# Autodesk Inventor assembly: Estrutura ax
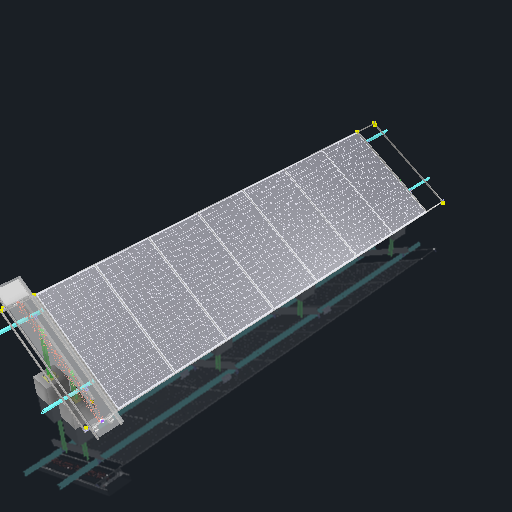
[picture p0: Inventor's stored thumbnail of the model, 512x512]
Saved by Autodesk Inventor 2025.3 (Build 293356030, 356C)
## iProperties
Created: 2019-12-15
Part Number: Estrutura ax
Document SubType Name: Assembly
Designer: Rubens
Sending System: SolidWorks 2021
Last Author: Mohsen
Last Saved: 2022-08-25
Author: Rubens
## Documents named in this file (17)
- C:\Users\Rubens\Downloads\Estrutura Placa - REV00\Solar Mounting Structure\Main_Solar_Structure\Main_Solar_Structure\Estrutura ax.iam
- C:\Users\Rubens\Downloads\Estrutura Placa - REV00\Solar Mounting Structure\Main_Solar_Structure\Main_Solar_Structure\Small_Column.ipt
- C:\Users\Rubens\Downloads\Estrutura Placa - REV00\Solar Mounting Structure\Main_Solar_Structure\Main_Solar_Structure\Large_Column.ipt
- C:\Users\Rubens\Downloads\Estrutura Placa - REV00\Solar Mounting Structure\Main_Solar_Structure\Main_Solar_Structure\Bottom_Beam.ipt
- C:\Users\Rubens\Downloads\Estrutura Placa - REV00\Solar Mounting Structure\Main_Solar_Structure\Main_Solar_Structure\Top_Beam.iam
- C:\Users\Rubens\Downloads\Estrutura Placa - REV00\Solar Mounting Structure\Main_Solar_Structure\Main_Solar_Structure\Base_Plate.ipt
- C:\Users\Rubens\Downloads\Estrutura Placa - REV00\Solar Mounting Structure\Main_Solar_Structure\Main_Solar_Structure\Base_Support.ipt
- C:\Users\Rubens\Downloads\Estrutura Placa - REV00\Solar Mounting Structure\Main_Solar_Structure\Main_Solar_Structure\Beam_Support.ipt
- C:\Users\Rubens\Downloads\Estrutura Placa - REV00\Solar Mounting Structure\Main_Solar_Structure\Main_Solar_Structure\M10_Screw&Nut.iam
- C:\Users\Rubens\Downloads\Estrutura Placa - REV00\Solar Mounting Structure\Main_Solar_Structure\Main_Solar_Structure\Beam_Connector_Assembly.iam
- C:\Users\Rubens\Downloads\Estrutura Placa - REV00\Solar Mounting Structure\Main_Solar_Structure\Main_Solar_Structure\Base.ipt
- C:\Users\Rubens\Downloads\Estrutura Placa - REV00\Solar Mounting Structure\Main_Solar_Structure\Main_Solar_Structure\ISO - 4034 - M16 - S_.ipt
- C:\Users\Rubens\Downloads\Limpador\MontagemREV0.iam
- C:\Users\Rubens\Downloads\Estrutura Placa - REV00\Solar Mounting Structure\Main_Solar_Structure\Main_Solar_Structure\SolarPV.ipt
- C:\Users\Rubens\Downloads\Estrutura Placa - REV00\Solar Mounting Structure\Main_Solar_Structure\Main_Solar_Structure\Perfil tubo - 30x30x3.ipt
- C:\Users\Rubens\Downloads\Estrutura Placa - REV00\Solar Mounting Structure\Main_Solar_Structure\Main_Solar_Structure\tubo 30 x 30 x 3  - 500.ipt
- C:\Users\Rubens\Downloads\Estrutura Placa - REV00\Solar Mounting Structure\Main_Solar_Structure\Main_Solar_Structure\Limitador.ipt
## Components (127 placed, 16 different names)
1. Small_Column:1 — Coincidente:18
2. Large_Column:1 — Coincidente:18
3. Bottom_Beam:1 — Coincidente:31, Coincidente:32, Coincidente:34
4. Bottom_Beam:2
5. Small_Column:2
6. Bottom_Beam:3
7. Small_Column:3
8. Bottom_Beam:4 — Coincidente:44, Coincidente:59
9. Small_Column:4
10. Top_Beam:3 [sub-assembly] — Coincidente:1, Coincidente:2, Coincidente:3, Coincidente:4, Coincidente:33, Alinhado:6, Coincidente:45
11. Top_Beam:4 [sub-assembly] — Coincidente:5, Coincidente:31, Coincidente:35, Alinhado:6, Coincidente:58
12. Base_Plate:1 — Coincidente:15
13. Base_Plate:2 — Coincidente:15, Coincidente:16, Coincidente:17
14. Base_Plate:4
15. Base_Plate:6
16. Base_Plate:8
17. Base_Support:1
18. Base_Support:2
19. Base_Support:3
20. Base_Support:7
21. Base_Support:8
22. Base_Support:9
23. Base_Support:13
24. Base_Support:14
25. Base_Support:15
26. Base_Support:19
27. Base_Support:20
28. Base_Support:21
29. Beam_Support:3 — Coincidente:32, Coincidente:33
30. Beam_Support:4 — Coincidente:34, Coincidente:35
31. Beam_Support:5
32. Beam_Support:6
33. Beam_Support:9
34. Beam_Support:10
35. M10_Screw&Nut:2 [sub-assembly]
36. M10_Screw&Nut:7 [sub-assembly]
37. M10_Screw&Nut:8 [sub-assembly]
38. M10_Screw&Nut:9 [sub-assembly]
39. M10_Screw&Nut:10 [sub-assembly]
40. M10_Screw&Nut:11 [sub-assembly]
41. M10_Screw&Nut:12 [sub-assembly]
42. M10_Screw&Nut:17 [sub-assembly]
43. M10_Screw&Nut:18 [sub-assembly]
44. M10_Screw&Nut:19 [sub-assembly]
45. M10_Screw&Nut:20 [sub-assembly]
46. M10_Screw&Nut:25 [sub-assembly]
47. M10_Screw&Nut:26 [sub-assembly]
48. M10_Screw&Nut:27 [sub-assembly]
49. M10_Screw&Nut:28 [sub-assembly]
50. M10_Screw&Nut:33 [sub-assembly]
51. M10_Screw&Nut:58 [sub-assembly] — Coincidente:62
52. M10_Screw&Nut:59 [sub-assembly] — Coincidente:63
53. M10_Screw&Nut:60 [sub-assembly]
54. M10_Screw&Nut:61 [sub-assembly]
55. M10_Screw&Nut:62 [sub-assembly]
56. M10_Screw&Nut:63 [sub-assembly]
57. M10_Screw&Nut:64 [sub-assembly]
58. M10_Screw&Nut:65 [sub-assembly]
59. M10_Screw&Nut:66 [sub-assembly]
60. M10_Screw&Nut:67 [sub-assembly]
61. M10_Screw&Nut:68 [sub-assembly]
62. M10_Screw&Nut:69 [sub-assembly]
63. M10_Screw&Nut:71 [sub-assembly] — Coincidente:60
64. M10_Screw&Nut:72 [sub-assembly] — Coincidente:61
65. M10_Screw&Nut:73 [sub-assembly]
66. M10_Screw&Nut:74 [sub-assembly]
67. M10_Screw&Nut:75 [sub-assembly]
68. M10_Screw&Nut:76 [sub-assembly]
69. M10_Screw&Nut:77 [sub-assembly]
70. M10_Screw&Nut:78 [sub-assembly]
71. M10_Screw&Nut:79 [sub-assembly]
72. M10_Screw&Nut:80 [sub-assembly]
73. M10_Screw&Nut:81 [sub-assembly]
74. Beam_Support:23 — Coincidente:44, Coincidente:45, Coincidente:62, Coincidente:63
75. Beam_Support:24
76. Beam_Support:25
77. Beam_Support:26 — Coincidente:58, Coincidente:59, Coincidente:60, Coincidente:61
78. Beam_Support:27
79. Beam_Support:28
80. M10_Screw&Nut:90 [sub-assembly]
81. M10_Screw&Nut:91 [sub-assembly]
82. Beam_Connector_Assembly:4 [sub-assembly]
83. Beam_Connector_Assembly:5 [sub-assembly]
84. Beam_Connector_Assembly:6 [sub-assembly]
85. Beam_Connector_Assembly:7 [sub-assembly]
86. Base:1 — Coincidente:13, Coincidente:14, Coincidente:16
87. Base:2 — Coincidente:13, Coincidente:14
88. ISO - 4034 - M16 - S_:2 — Coincidente:17
89. ISO - 4034 - M16 - S_:43
90. ISO - 4034 - M16 - S_:47
91. ISO - 4034 - M16 - S_:51
92. ISO - 4034 - M16 - S_:55
93. ISO - 4034 - M16 - S_:48
94. ISO - 4034 - M16 - S_:44
95. ISO - 4034 - M16 - S_:56
96. ISO - 4034 - M16 - S_:52
97. Base:4
98. ISO - 4034 - M16 - S_:50
99. ISO - 4034 - M16 - S_:46
100. ISO - 4034 - M16 - S_:58
101. ISO - 4034 - M16 - S_:54
102. Base:6
103. ISO - 4034 - M16 - S_:49
104. ISO - 4034 - M16 - S_:45
105. ISO - 4034 - M16 - S_:57
106. ISO - 4034 - M16 - S_:53
107. Base:8
108. MontagemREV0:1 [sub-assembly] — Alinhado:1, Coincidente:6, Coincidente:25
109. SolarPV:1 — Coincidente:1, Alinhado:1, Coincidente:6, Coincidente:19, Coincidente:20, Coincidente:25, Coincidente:42, Coincidente:43
110. SolarPV:2 — Coincidente:2, Coincidente:19, Coincidente:20, Coincidente:21, Coincidente:22
111. SolarPV:3 — Coincidente:3, Coincidente:21, Coincidente:22, Coincidente:23, Coincidente:24
112. SolarPV:4 — Coincidente:4, Coincidente:7, Coincidente:8, Coincidente:23, Coincidente:24
113. SolarPV:5 — Coincidente:5, Coincidente:7, Coincidente:8, Coincidente:9, Coincidente:10
114. SolarPV:6 — Coincidente:9, Coincidente:10, Coincidente:11, Coincidente:12
115. SolarPV:7 — Coincidente:11, Coincidente:12, Coincidente:51, Coincidente:52
116. Perfil tubo - 30x30x3:1 — Coincidente:42, Coincidente:43
117. Perfil tubo - 30x30x3:2 — Coincidente:54, Coincidente:55, Coincidente:56
118. tubo 30 x 30 x 3  - 500:1
119. tubo 30 x 30 x 3  - 500:2 — Coincidente:53
120. Perfil tubo - 30x30x3:3 — Coincidente:64, Coincidente:65
121. Perfil tubo - 30x30x3:4 — Coincidente:51
122. tubo 30 x 30 x 3  - 500:3 — Coincidente:52
123. tubo 30 x 30 x 3  - 500:4 — Coincidente:57
124. Limitador:1 — Coincidente:53, Coincidente:54
125. Limitador:2 — Coincidente:55, Coincidente:56
126. Limitador:3 — Coincidente:57
127. Limitador:4 — Coincidente:64, Coincidente:65
## Relationships (69: Mate 59, Flush 10)
- Coincidente:1 [Mate]: Top_Beam:3 ↔ SolarPV:1
- Coincidente:2 [Mate]: Top_Beam:3 ↔ SolarPV:2
- Coincidente:3 [Mate]: Top_Beam:3 ↔ SolarPV:3
- Coincidente:4 [Mate]: Top_Beam:3 ↔ SolarPV:4
- Coincidente:5 [Mate]: Top_Beam:4 ↔ SolarPV:5
- Alinhado:1 [Flush] (-550 mm): MontagemREV0:1 ↔ SolarPV:1
- Coincidente:6 [Mate] (50 mm): MontagemREV0:1 ↔ SolarPV:1
- Coincidente:7 [Mate]: SolarPV:4 ↔ SolarPV:5
- Coincidente:8 [Mate]: SolarPV:4 ↔ SolarPV:5
- Coincidente:9 [Mate]: SolarPV:5 ↔ SolarPV:6
- Coincidente:10 [Mate]: SolarPV:5 ↔ SolarPV:6
- Coincidente:11 [Mate]: SolarPV:6 ↔ SolarPV:7
- Coincidente:12 [Mate]: SolarPV:6 ↔ SolarPV:7
- Coincidente:13 [Mate] (300 mm): Base:1 ↔ Base:2
- Coincidente:14 [Mate]: Base:1 ↔ Base:2
- Coincidente:15 [Mate]: Base_Plate:1 ↔ Base_Plate:2
- Coincidente:16 [Mate]: Base_Plate:2 ↔ Base:1
- Coincidente:17 [Mate]: Base_Plate:2 ↔ ISO - 4034 - M16 - S_:2
- Coincidente:18 [Mate] (600 mm): Small_Column:1 ↔ Large_Column:1
- Coincidente:19 [Mate]: SolarPV:1 ↔ SolarPV:2
- Coincidente:20 [Mate]: SolarPV:1 ↔ SolarPV:2
- Coincidente:21 [Mate]: SolarPV:2 ↔ SolarPV:3
- Coincidente:22 [Mate]: SolarPV:2 ↔ SolarPV:3
- Coincidente:23 [Mate]: SolarPV:3 ↔ SolarPV:4
- Coincidente:24 [Mate]: SolarPV:3 ↔ SolarPV:4
- Coincidente:25 [Mate]: MontagemREV0:1 ↔ SolarPV:1
- [Mate]: Perfil tubo - 30x30x3:1 ↔ tubo 30 x 30 x 3  - 500:2
- [Mate]: Perfil tubo - 30x30x3:1 ↔ tubo 30 x 30 x 3  - 500:1
- [Flush]: Perfil tubo - 30x30x3:1 ↔ tubo 30 x 30 x 3  - 500:1
- [Flush]: Perfil tubo - 30x30x3:1 ↔ tubo 30 x 30 x 3  - 500:1
- [Mate]: Perfil tubo - 30x30x3:2 ↔ tubo 30 x 30 x 3  - 500:1
- [Flush]: Perfil tubo - 30x30x3:2 ↔ tubo 30 x 30 x 3  - 500:1
- [Mate]: Perfil tubo - 30x30x3:2 ↔ tubo 30 x 30 x 3  - 500:1
- [Mate]: Perfil tubo - 30x30x3:1 ↔ tubo 30 x 30 x 3  - 500:2
- [Flush]: Perfil tubo - 30x30x3:1 ↔ tubo 30 x 30 x 3  - 500:2
- Coincidente:31 [Mate]: Bottom_Beam:1 ↔ Top_Beam:4
- Coincidente:32 [Mate]: Bottom_Beam:1 ↔ Beam_Support:3
- Coincidente:33 [Mate]: Top_Beam:3 ↔ Beam_Support:3
- Coincidente:34 [Mate]: Bottom_Beam:1 ↔ Beam_Support:4
- Coincidente:35 [Mate]: Top_Beam:4 ↔ Beam_Support:4
- Alinhado:6 [Flush]: Top_Beam:3 ↔ Top_Beam:4
- Coincidente:42 [Mate]: SolarPV:1 ↔ Perfil tubo - 30x30x3:1
- Coincidente:43 [Mate]: SolarPV:1 ↔ Perfil tubo - 30x30x3:1
- Coincidente:44 [Mate]: Bottom_Beam:4 ↔ Beam_Support:23
- Coincidente:45 [Mate]: Top_Beam:3 ↔ Beam_Support:23
- [Mate]: Perfil tubo - 30x30x3:3 ↔ tubo 30 x 30 x 3  - 500:4
- [Mate]: Perfil tubo - 30x30x3:3 ↔ tubo 30 x 30 x 3  - 500:3
- [Flush]: Perfil tubo - 30x30x3:3 ↔ tubo 30 x 30 x 3  - 500:3
- [Flush]: Perfil tubo - 30x30x3:3 ↔ tubo 30 x 30 x 3  - 500:3
- [Mate]: Perfil tubo - 30x30x3:4 ↔ tubo 30 x 30 x 3  - 500:3
- [Flush]: Perfil tubo - 30x30x3:4 ↔ tubo 30 x 30 x 3  - 500:3
- [Mate]: Perfil tubo - 30x30x3:4 ↔ tubo 30 x 30 x 3  - 500:3
- [Mate]: Perfil tubo - 30x30x3:3 ↔ tubo 30 x 30 x 3  - 500:4
- [Flush]: Perfil tubo - 30x30x3:3 ↔ tubo 30 x 30 x 3  - 500:4
- Coincidente:51 [Mate]: SolarPV:7 ↔ Perfil tubo - 30x30x3:4
- Coincidente:52 [Mate]: SolarPV:7 ↔ tubo 30 x 30 x 3  - 500:3
- Coincidente:53 [Mate]: tubo 30 x 30 x 3  - 500:2 ↔ Limitador:1
- Coincidente:54 [Mate]: Perfil tubo - 30x30x3:2 ↔ Limitador:1
- Coincidente:55 [Mate]: Perfil tubo - 30x30x3:2 ↔ Limitador:2
- Coincidente:56 [Mate]: Perfil tubo - 30x30x3:2 ↔ Limitador:2
- Coincidente:57 [Mate]: tubo 30 x 30 x 3  - 500:4 ↔ Limitador:3
- Coincidente:58 [Mate]: Top_Beam:4 ↔ Beam_Support:26
- Coincidente:59 [Mate]: Bottom_Beam:4 ↔ Beam_Support:26
- Coincidente:60 [Mate]: M10_Screw&Nut:71 ↔ Beam_Support:26
- Coincidente:61 [Mate]: M10_Screw&Nut:72 ↔ Beam_Support:26
- Coincidente:62 [Mate]: M10_Screw&Nut:58 ↔ Beam_Support:23
- Coincidente:63 [Mate]: M10_Screw&Nut:59 ↔ Beam_Support:23
- Coincidente:64 [Mate]: Perfil tubo - 30x30x3:3 ↔ Limitador:4
- Coincidente:65 [Mate]: Perfil tubo - 30x30x3:3 ↔ Limitador:4
## Named parameters: d92_d72 = 0 mm, d93_d73 = 0 mm, d94_d74 = 0 mm, d95_d75 = 0 mm, d96_d76 = 0 mm, d97_d77 = 0 mm, d98_d79 = 0 mm, d99_d80 = 0 mm, d100_d81 = 0 mm
